# Autodesk Inventor assembly: 頭組
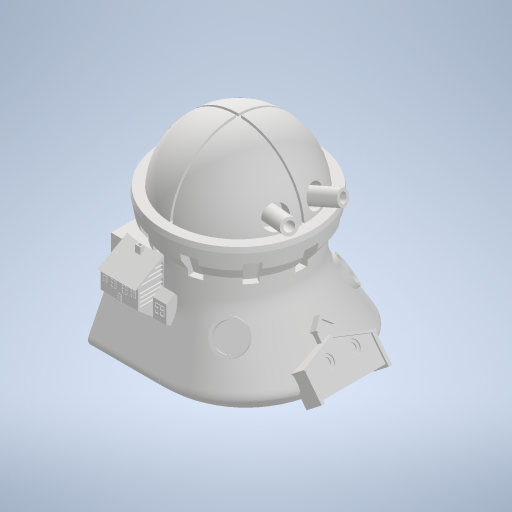
[picture p0: Inventor's stored thumbnail of the model, 512x512]
Saved by Autodesk Inventor 2024 (Build 280153000, 153)
## iProperties
Created: 2024-05-22
Part Number: 頭組
Document SubType Name: Assembly
Designer: User
Author: User
## Documents named in this file (5)
- C:\Users\User\Documents\Inventor\construction\頭組.iam
- C:\Users\User\Documents\Inventor\construction\屋頂-3.ipt
- C:\Users\User\Documents\Inventor\construction\頭改.ipt
- C:\Users\User\Documents\Inventor\construction\屋-2 物1.ipt
- C:\Users\User\Documents\Inventor\construction\頭 小小屋.ipt
## Components (4 placed, 4 different names)
1. 屋頂-3:1 — 貼合:1, 貼合:2
2. 頭改:1 — 貼合:1, 貼合:2, 齊平:1, 貼合:3
3. 屋-2 物1:1 — 齊平:1
4. 頭 小小屋:1 — 貼合:3
## Relationships (4: Mate 3, Flush 1)
- 貼合:1 [Mate]: 屋頂-3:1 ↔ 頭改:1
- 貼合:2 [Mate]: 屋頂-3:1 ↔ 頭改:1
- 齊平:1 [Flush] (-10 mm): 頭改:1 ↔ 屋-2 物1:1
- 貼合:3 [Mate]: 頭改:1 ↔ 頭 小小屋:1
